# Autodesk Inventor assembly: Ensamblaje5
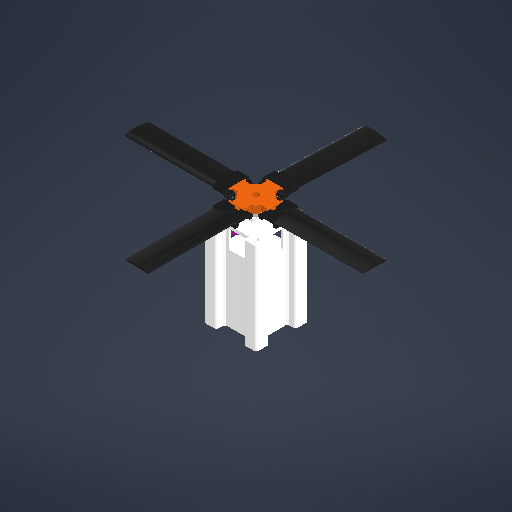
[picture p0: Inventor's stored thumbnail of the model, 512x512]
Saved by Autodesk Inventor 2026.1 (Build 301233000, 233)
## iProperties
Created: 2025-11-12
Part Number: Ensamblaje5
Document SubType Name: Assembly
Designer: usuario
Mass: 926.641 g
Surface Area: 2833.49 cm^2
Volume: 714.155 cm^3
Density: 1.29753 g/cm^3
Author: usuario
## Documents named in this file (9)
- C:\Users\usuario\Documents\vickh_Cansat\Cansat_Huitzilin\3D\NuevoDiseno\Ensamblaje5.iam
- C:\Users\usuario\Documents\vickh_Cansat\Cansat_Huitzilin\3D\NuevoDiseno\Electronica.ipt
- C:\Users\usuario\Documents\vickh_Cansat\Cansat_Huitzilin\3D\NuevoDiseno\SubSistemaLiberacion.iam
- C:\Users\usuario\Documents\vickh_Cansat\Cansat_Huitzilin\3D\NuevoDiseno\Ensamblaje5\AIP\FEA\f8yce27ts.fins
- C:\Users\usuario\Documents\vickh_Cansat\Cansat_Huitzilin\3D\NuevoDiseno\Ensamblaje5\AIP\FEA\f8yce27ts.fsat
- C:\Users\usuario\Documents\vickh_Cansat\Cansat_Huitzilin\3D\NuevoDiseno\Ensamblaje5\AIP\FEA\f8yce27ts.ftes
- C:\Users\usuario\Documents\vickh_Cansat\Cansat_Huitzilin\3D\NuevoDiseno\Ensamblaje5\AIP\FEA\f8yce27ts.fwiz
- C:\Users\usuario\Documents\vickh_Cansat\Cansat_Huitzilin\3D\NuevoDiseno\Ensamblaje5\AIP\FEA\f8yce27vk.fmsh
- C:\Users\usuario\Documents\vickh_Cansat\Cansat_Huitzilin\3D\NuevoDiseno\Ensamblaje5\AIP\FEA\f8yce27vl.fres
## Components (2 placed, 2 different names)
1. Electronica:1
2. SubSistemaLiberacion:1 [sub-assembly]
## Named parameters: sa_0 = 0, sa_1 = -981, sa_2 = 0, sa_3 = 1.5e+06
note: some values were not read from the file. Shown as the stored number, unit unknown: "sa_0", "sa_1", "sa_2", "sa_3".
